# Autodesk Inventor assembly: Servo 180 Degree
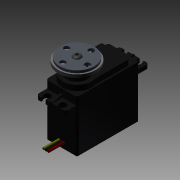
[picture p0: Inventor's stored thumbnail of the model, 180x180]
Saved by Autodesk Inventor 2015 (Build 190159000, 159)
## iProperties
Created: 2015-10-21
Part Number: Servo 180 Degree
Document SubType Name: Assembly
Designer: Mason
Author: Mason
## Documents named in this file (5)
- C:\Users\Mason\Documents\Inventor\Content Center Files\FTC\Servo 180 Degree.iam
- C:\Users\Mason\Documents\Inventor\Content Center Files\FTC\Servo 180 Degree .asm Parts\Servo 180 Degree  Servo.ipt
- C:\Users\Mason\Documents\Inventor\Content Center Files\FTC\Servo 180 Degree .asm Parts\Servo 180 Degree Metal Horn.ipt
- C:\Users\Mason\Documents\Inventor\Content Center Files\FTC\Servo 180 Degree .asm Parts\Servo 180 Degree Screw.ipt
- C:\Users\Mason\Documents\Inventor\Content Center Files\FTC\Servo 180 Degree .asm Parts\Servo 180 Degree Plasitc Horn.ipt
## Components (5 placed, 4 different names)
1. Servo 180 Degree  Servo:1 — Insert:1
2. Servo 180 Degree Metal Horn:1 — Insert:4
3. Servo 180 Degree Screw:1 — Insert:2, Insert:4
4. Servo 180 Degree Plasitc Horn:1 — Insert:3
5. Servo 180 Degree Screw:2 — Insert:1, Insert:2, Insert:3
## Relationships (4: Insert 4)
- Insert:1 (-7 mm): Servo 180 Degree  Servo:1 ↔ Servo 180 Degree Screw:2
- Insert:2 (-8 mm): Servo 180 Degree Screw:1 ↔ Servo 180 Degree Screw:2
- Insert:3: Servo 180 Degree Plasitc Horn:1 ↔ Servo 180 Degree Screw:2
- Insert:4: Servo 180 Degree Metal Horn:1 ↔ Servo 180 Degree Screw:1
